# Autodesk Inventor assembly: Assembly_Cube_explosion_v2
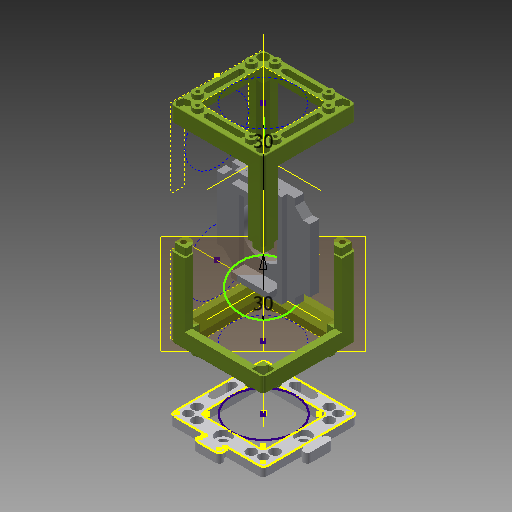
[picture p0: Inventor's stored thumbnail of the model, 512x512]
Saved by Autodesk Inventor 2019 (Build 230136000, 136)
## iProperties
Created: 2020-03-27
Part Number: Assembly_Cube_explosion_v2
Document SubType Name: Assembly
Designer: B
Author: B
## Documents named in this file (5)
- C:\Users\UC2\Dropbox\UC2\02_CAD\INVENTOR\uc2_v3\Assembly_Cube_explosion_IM_v3.iam
- C:\Users\UC2\Dropbox\UC2\02_CAD\INVENTOR\uc2_v3\20_Cube_Insert_Sample_clamp.ipt
- C:\Users\UC2\Dropbox\UC2\02_CAD\INVENTOR\uc2_v3\20_Cube_insert_Sample_holder_v3.ipt
- C:\Users\UC2\Dropbox\UC2\02_CAD\INVENTOR\uc2_v3\10_Base_puzzle_v3.ipt
- C:\Users\UC2\Dropbox\UC2\02_CAD\INVENTOR\uc2_v3\10_Cube_1x1_IM.ipt
## Components (5 placed, 4 different names)
1. 10_Base_puzzle_v3:1 — Mate:18, Angle:4, Mate:19, Mate:20
2. 10_Cube_1x1_IM:1 — Mate:15, Mate:16, Mate:17, Flush:5
3. 10_Cube_1x1_IM:2 — Mate:17, Flush:5, Angle:3, Mate:18, Angle:4
4. 20_Cube_Insert_Sample_clamp:1 — Mate:13, Mate:14, Flush:4
5. 20_Cube_insert_Sample_holder_v3:1 — Mate:13, Mate:14, Flush:4, Mate:15, Angle:3, Mate:16
## Relationships (14: Mate 9, Angle 3, Flush 2)
- [Mate]: 10_Cube_1x1_IM:1 ↔ 10_Cube_1x1_IM:2
- [Angle] (0 deg): 10_Cube_1x1_IM:1 ↔ 10_Cube_1x1_IM:2
- Mate:13: 20_Cube_Insert_Sample_clamp:1 ↔ 20_Cube_insert_Sample_holder_v3:1
- Mate:14: 20_Cube_Insert_Sample_clamp:1 ↔ 20_Cube_insert_Sample_holder_v3:1
- Flush:4: 20_Cube_Insert_Sample_clamp:1 ↔ 20_Cube_insert_Sample_holder_v3:1
- Mate:15: 10_Cube_1x1_IM:1 ↔ 20_Cube_insert_Sample_holder_v3:1
- Angle:3 (0 deg): 10_Cube_1x1_IM:2 ↔ 20_Cube_insert_Sample_holder_v3:1
- Mate:16: 10_Cube_1x1_IM:1 ↔ 20_Cube_insert_Sample_holder_v3:1
- Mate:17: 10_Cube_1x1_IM:1 ↔ 10_Cube_1x1_IM:2
- Flush:5: 10_Cube_1x1_IM:1 ↔ 10_Cube_1x1_IM:2
- Mate:18: 10_Base_puzzle_v3:1 ↔ 10_Cube_1x1_IM:2
- Angle:4 (0 deg): 10_Base_puzzle_v3:1 ↔ 10_Cube_1x1_IM:2
- Mate:19: 10_Base_puzzle_v3:1
- Mate:20: 10_Base_puzzle_v3:1
